# Autodesk Inventor assembly: shootingMechanism
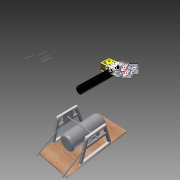
[picture p0: Inventor's stored thumbnail of the model, 180x180]
Saved by Autodesk Inventor 2014 SP2 (Build 180246200, 246)
## iProperties
Created: 2016-04-20
Part Number: shootingMechanism
Document SubType Name: Assembly
Designer: Administrator
Author: Administrator
## Documents named in this file (17)
- Z:\RoboEaglesCAD\TShirty5\shootingMechanism.iam
- Z:\RoboEaglesCAD\TShirty5\woodPlate.ipt
- Z:\RoboEaglesCAD\TShirty5\daGasContiner.ipt
- Z:\RoboEaglesCAD\TShirty5\16inSquarePipe.ipt
- Z:\RoboEaglesCAD\TShirty5\10inSquarePipe.ipt
- Z:\RoboEaglesCAD\TShirty5\Wonkey.ipt
- Z:\RoboEaglesCAD\TShirty5\mountingPanelCannon.ipt
- Z:\RoboEaglesCAD\TShirty5\midBrace.ipt
- Z:\RoboEaglesCAD\TShirty5\bigShaft2.ipt
- Z:\RoboEaglesCAD\TShirty5\Imported Components\Solenoid\Solenoid.ipt
- Z:\RoboEaglesCAD\TShirty5\Cannon.ipt
- Z:\RoboEaglesCAD\TShirty5\Cap.ipt
- Z:\RoboEaglesCAD\TShirty5\CapSleeve.ipt
- Z:\RoboEaglesCAD\TShirty5\Holder.ipt
- Z:\RoboEaglesCAD\TShirty5\Strap.ipt
- Z:\RoboEaglesCAD\TShirty5\Imported Components\Bolt4inch10-32\Bolt4inch10-32.ipt
- Z:\RoboEaglesCAD\TShirty5\Imported Components\am-2568 500EX Hex Hub\am-2568 500EX Hex Hub.ipt
## Components (31 placed, 16 different names)
1. woodPlate:1 — Tangent:1, Flush:1, Flush:6, Flush:7, Mate:5, Mate:13
2. daGasContiner:1 — Tangent:1
3. 16inSquarePipe:3 — Mate:12, Mate:13, Mate:15, Flush:12, Mate:16
4. 16inSquarePipe:4 — Flush:8, Mate:5, Mate:6, Mate:8, Mate:9, Flush:11, Mate:18
5. 10inSquarePipe:1 — Flush:7, Flush:8, Mate:7, Flush:9, Mate:10, Mate:11, Flush:14, Flush:15, Mate:20, Flush:19, Flush:23, Flush:29
6. 10inSquarePipe:2 — Flush:6, Mate:14, Flush:13, Mate:17, Flush:14, Mate:19, Flush:16, Flush:22, Mate:21, Flush:26
7. Wonkey:1 — Mate:8, Mate:9, Flush:9
8. Wonkey:2 — Mate:16, Flush:13, Mate:17
9. Wonkey:3 — Flush:11, Mate:10, Mate:11, Mate:18, Flush:15, Mate:23, Flush:27
10. Wonkey:4 — Mate:12, Mate:14, Mate:15, Flush:12, Mate:19, Flush:16, Mate:22, Flush:24
11. mountingPanelCannon:2 — Mate:20, Flush:19, Flush:23, Flush:28, Flush:29, Mate:25
12. mountingPanelCannon:4 — Flush:22, Mate:21, Flush:25, Flush:26, Mate:24
13. midBrace:1 — Mate:23, Flush:27, Flush:28
14. midBrace:2 — Mate:22, Flush:24, Flush:25
15. bigShaft2:1 — Mate:24, Mate:26, Angle:1
16. bigShaft2:2 — Mate:25, Mate:26, Angle:1, Mate:27, Mate:28
17. bigShaft2:1 — Mate:27, Mate:28
18. Solenoid:1 — Insert:3
19. Cannon:1 — Insert:1, Mate:29, Mate:33, Mate:34
20. Cap:1 — Insert:1, Insert:2, Insert:3
21. CapSleeve:1 — Insert:2, Mate:30
22. Holder:1 — Mate:29, Mate:30, Mate:31, Mate:32, Flush:30, Flush:31, Mate:35, Mate:36, Mate:37
23. Strap:1 — Mate:32, Mate:33, Flush:31
24. Strap:2 — Mate:31, Mate:34, Flush:30
25. Bolt4inch10-32:1
26. am-2568 500EX Hex Hub:1 — Mate:36, Mate:37, Mate:38
27. am-2568 500EX Hex Hub:2 — Mate:35
28. Bolt4inch10-32:2
29. Bolt4inch10-32:3
30. Bolt4inch10-32:4
31. Bolt4inch10-32:5
## Relationships (61: Mate 34, Flush 22, Insert 3, Tangent 1, Angle 1)
- Tangent:1: woodPlate:1 ↔ daGasContiner:1
- Flush:1 (190.5 mm): woodPlate:1
- Flush:6: woodPlate:1 ↔ 10inSquarePipe:2
- Flush:7: woodPlate:1 ↔ 10inSquarePipe:1
- Flush:8 (-76.2 mm): 16inSquarePipe:4 ↔ 10inSquarePipe:1
- Mate:5: woodPlate:1 ↔ 16inSquarePipe:4
- Mate:6: 16inSquarePipe:4
- Mate:7: 10inSquarePipe:1
- Mate:8: 16inSquarePipe:4 ↔ Wonkey:1
- Mate:9: 16inSquarePipe:4 ↔ Wonkey:1
- Flush:9: 10inSquarePipe:1 ↔ Wonkey:1
- Flush:11: 16inSquarePipe:4 ↔ Wonkey:3
- Mate:10: 10inSquarePipe:1 ↔ Wonkey:3
- Mate:11: 10inSquarePipe:1 ↔ Wonkey:3
- Mate:12: 16inSquarePipe:3 ↔ Wonkey:4
- Mate:13: woodPlate:1 ↔ 16inSquarePipe:3
- Mate:14: 10inSquarePipe:2 ↔ Wonkey:4
- Mate:15: 16inSquarePipe:3 ↔ Wonkey:4
- Flush:12: 16inSquarePipe:3 ↔ Wonkey:4
- Mate:16: 16inSquarePipe:3 ↔ Wonkey:2
- Flush:13: 10inSquarePipe:2 ↔ Wonkey:2
- Mate:17: 10inSquarePipe:2 ↔ Wonkey:2
- Flush:14: 10inSquarePipe:1 ↔ 10inSquarePipe:2
- Mate:18: 16inSquarePipe:4 ↔ Wonkey:3
- Flush:15: 10inSquarePipe:1 ↔ Wonkey:3
- Mate:19: 10inSquarePipe:2 ↔ Wonkey:4
- Flush:16: 10inSquarePipe:2 ↔ Wonkey:4
- Mate:20: 10inSquarePipe:1 ↔ mountingPanelCannon:2
- Flush:19 (63.5 mm): 10inSquarePipe:1 ↔ mountingPanelCannon:2
- Flush:22 (63.5 mm): 10inSquarePipe:2 ↔ mountingPanelCannon:4
- Mate:21: 10inSquarePipe:2 ↔ mountingPanelCannon:4
- Flush:23: 10inSquarePipe:1 ↔ mountingPanelCannon:2
- Mate:22: Wonkey:4 ↔ midBrace:2
- Flush:24: Wonkey:4 ↔ midBrace:2
- Flush:25: mountingPanelCannon:4 ↔ midBrace:2
- Flush:26: 10inSquarePipe:2 ↔ mountingPanelCannon:4
- Mate:23: Wonkey:3 ↔ midBrace:1
- Flush:27: Wonkey:3 ↔ midBrace:1
- Flush:28: mountingPanelCannon:2 ↔ midBrace:1
- Flush:29: 10inSquarePipe:1 ↔ mountingPanelCannon:2
- Mate:24: mountingPanelCannon:4 ↔ bigShaft2:1
- Mate:25: mountingPanelCannon:2 ↔ bigShaft2:2
- Mate:26: bigShaft2:1 ↔ bigShaft2:2
- Angle:1 (0 deg): bigShaft2:1 ↔ bigShaft2:2
- Mate:27: bigShaft2:2 ↔ bigShaft2:1
- Mate:28: bigShaft2:2 ↔ bigShaft2:1
- Insert:1: Cannon:1 ↔ Cap:1
- Insert:2: Cap:1 ↔ CapSleeve:1
- Insert:3: Solenoid:1 ↔ Cap:1
- Mate:29: Cannon:1 ↔ Holder:1
- Mate:30: CapSleeve:1 ↔ Holder:1
- Mate:31: Holder:1 ↔ Strap:2
- Mate:32: Holder:1 ↔ Strap:1
- Mate:33: Cannon:1 ↔ Strap:1
- Mate:34: Cannon:1 ↔ Strap:2
- Flush:30: Holder:1 ↔ Strap:2
- Flush:31: Holder:1 ↔ Strap:1
- Mate:35: Holder:1 ↔ am-2568 500EX Hex Hub:2
- Mate:36: Holder:1 ↔ am-2568 500EX Hex Hub:1
- Mate:37: Holder:1 ↔ am-2568 500EX Hex Hub:1
- Mate:38: am-2568 500EX Hex Hub:1
